# Autodesk Inventor assembly: Distribution module
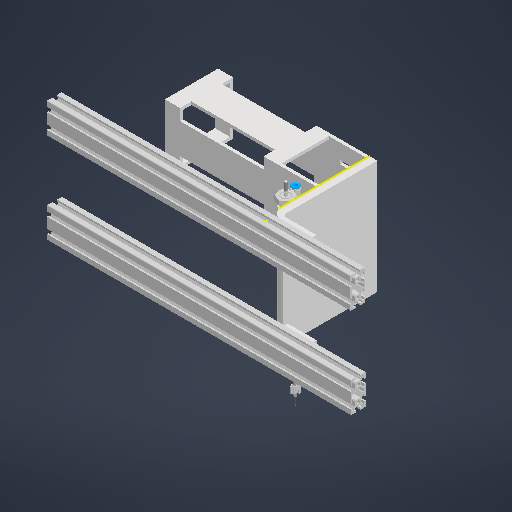
[picture p0: Inventor's stored thumbnail of the model, 512x512]
Saved by Autodesk Inventor 2027 (Build 310192000, 192)
## iProperties
Created: 2026-04-16
Part Number: Distribution module
Document SubType Name: Assembly
Designer: ratik
Author: ratik
## Documents named in this file (4)
- C:\Users\ratik\OneDrive\Personal Folder\00_Startup\01_Mectosys_Prototype\01_Prototype\01_Mechanical\3D file\Assembly File\Distribution module.iam
- C:\Users\ratik\OneDrive\Personal Folder\00_Startup\01_Mectosys_Prototype\01_Prototype\01_Mechanical\3D file\02_Slider\10_HFS5-2040-1500_Inventor\HFS5-2040-1500.ipt
- C:\Users\ratik\OneDrive\Personal Folder\00_Startup\01_Mectosys_Prototype\01_Prototype\01_Mechanical\3D file\04_Distribution module\44_Housing\Housing.ipt
- C:\Users\ratik\OneDrive\Personal Folder\00_Startup\01_Mectosys_Prototype\01_Prototype\01_Mechanical\3D file\04_Distribution module\Cylinder assembly\cylinder assembly.iam
## Components (4 placed, 3 different names)
1. HFS5-2040-1500:1 — Mate:1
2. Housing:1 — Mate:1, Mate:2, Flush:1
3. HFS5-2040-1500:2 — Mate:2
4. cylinder assembly:1 [sub-assembly] — Flush:1
## Relationships (3: Mate 2, Flush 1)
- Mate:1: HFS5-2040-1500:1 ↔ Housing:1
- Mate:2: Housing:1 ↔ HFS5-2040-1500:2
- Flush:1: Housing:1 ↔ cylinder assembly:1
